# Autodesk Inventor assembly: Assembly1
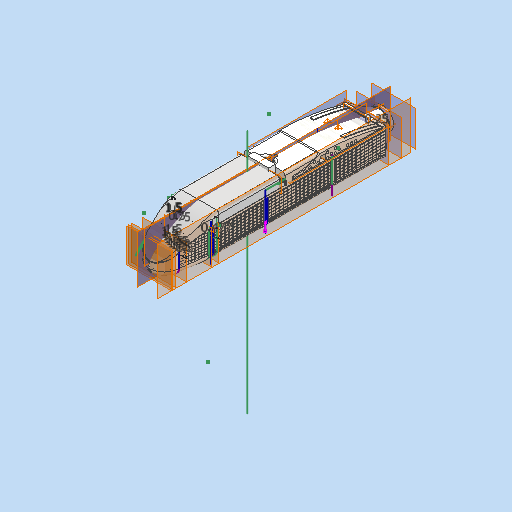
[picture p0: Inventor's stored thumbnail of the model, 512x512]
Saved by Autodesk Inventor 2027 (Build 310192060, 192F)
## iProperties
Created: 2026-08-07
Part Number: Assembly1
Document SubType Name: Assembly
Designer: mateo
Author: mateo
## Documents named in this file (5)
- C:\GitHub\SWIFT-UAV\System_development\Pelican\structural_model\v0.3.0\Parts\STEP\Assembly1.iam
- C:\GitHub\SWIFT-UAV\System_development\Pelican\structural_model\v0.3.0\Parts\Wings\WingBox.ipt
- C:\GitHub\SWIFT-UAV\System_development\Pelican\structural_model\v0.3.1\Parts\Fuselage\FuselageV2.ipt
- C:\GitHub\SWIFT-UAV\System_development\Pelican\structural_model\v0.3.0\Parts\Cover\FrontCover.ipt
- C:\GitHub\SWIFT-UAV\System_development\Pelican\structural_model\v0.3.1\Parts\Ancillary Components\MotorHousingV2.ipt
## Components (4 placed, 4 different names)
1. WingBox:1 — Mate:1
2. FuselageV2:1 — Mate:1, Mate:2, Mate:3, Mate:4, Mate:5, Mate:6
3. FrontCover:1 — Mate:2, Mate:3
4. MotorHousingV2:1 — Mate:4, Mate:5, Mate:6
## Relationships (6: Mate 6)
- Mate:1: WingBox:1 ↔ FuselageV2:1
- Mate:2: FuselageV2:1 ↔ FrontCover:1
- Mate:3: FuselageV2:1 ↔ FrontCover:1
- Mate:4: FuselageV2:1 ↔ MotorHousingV2:1
- Mate:5: FuselageV2:1 ↔ MotorHousingV2:1
- Mate:6: FuselageV2:1 ↔ MotorHousingV2:1
